# Autodesk Inventor assembly: mount3
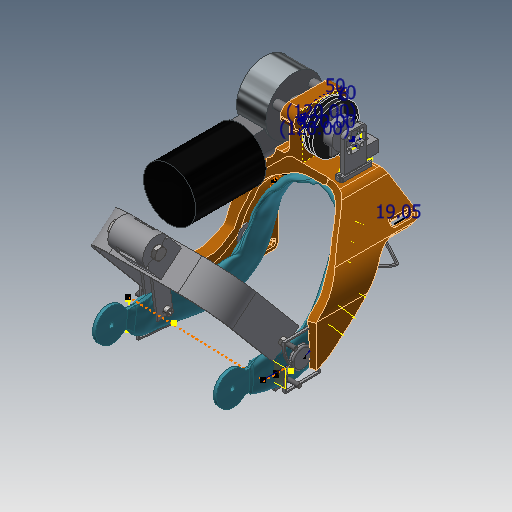
[picture p0: Inventor's stored thumbnail of the model, 512x512]
Saved by Autodesk Inventor 2025.2 (Build 292293000, 293)
## iProperties
Created: 2025-02-11
Part Number: mount3
Document SubType Name: Assembly
Designer: Alex
Author: Alex
## Documents named in this file (13)
- C:\Users\email\Desktop\Projects\Capstone\4TB6\CAD_Model\thigh_mount_2\mount3.iam
- C:\Users\email\Desktop\Projects\Capstone\4TB6\CAD_Model\thigh_mount_2\thigh.ipt
- C:\Users\email\Desktop\Projects\Capstone\4TB6\CAD_Model\thigh_mount_2\mount3.ipt
- C:\Users\email\Desktop\Projects\Capstone\4TB6\CAD_Model\thigh_mount_2\mount4.ipt
- C:\Users\email\Desktop\Projects\Capstone\4TB6\CAD_Model\thigh_mount_2\motor.ipt
- C:\Users\email\Desktop\Projects\Capstone\4TB6\CAD_Model\thigh_mount_2\spool_temp.ipt
- C:\Users\email\Desktop\Projects\Capstone\4TB6\CAD_Model\thigh_mount_2\magnetholder.ipt
- C:\Users\email\Desktop\Projects\Capstone\4TB6\CAD_Model\thigh_mount_2\imu_house_assembly.iam
- C:\Users\email\Desktop\Projects\Capstone\4TB6\CAD_Model\thigh_mount_2\ANSI B18.6.7M - M6x1 x 13(6).ipt
- C:\Users\email\Desktop\Projects\Capstone\4TB6\CAD_Model\thigh_mount_2\as5600mount_2.ipt
- C:\Users\email\Desktop\Projects\Capstone\4TB6\CAD_Model\thigh_mount_2\pulley_bracket_assem.iam
- C:\Users\email\Desktop\Projects\Capstone\4TB6\CAD_Model\thigh_mount_2\brace_tabs.ipt
- C:\Users\email\Desktop\Projects\Capstone\4TB6\CAD_Model\thigh_mount_2\brace_tabs_half.ipt
## Components (14 placed, 12 different names)
1. thigh:1 — Mate:1, Mate:2, Flush:1, Flush:2, Mate:28, Mate:29, Mate:30, Mate:31, Mate:32, Mate:33, Mate:34
2. mount3:1 — Flush:2
3. mount4:1 — Flush:4, Mate:3, Mate:4, Mate:5, Mate:12, Mate:13, Flush:5, Angle:7, Angle:2, Mate:21, Mate:22, Mate:27
4. motor:1 — Mate:3, Mate:4, Mate:5, Mate:7, Mate:23, Mate:24
5. spool_temp:1 — Mate:7, Mate:9, Mate:10, Mate:11, Mate:23, Mate:24
6. magnetholder:1 — Mate:9, Mate:10, Mate:11, Mate:18, Mate:25, Mate:26
7. imu_house_assembly:1 [sub-assembly] — Mate:12, Mate:13, Flush:5, Mate:14, Mate:15
8. Square Recessed Pan Head Machine Screw - Type III - Metric M6x1 x 13:1 — Mate:14, Mate:15
9. as5600mount_2:1 — Mate:18, Mate:25, Mate:26, Mate:27
10. pulley_bracket_assem:1 [sub-assembly] — Angle:7, Angle:2, Mate:21, Mate:22
11. brace_tabs:1 — Mate:28, Mate:29
12. brace_tabs:2 — Mate:30, Mate:31
13. brace_tabs_half:1 — Mate:32
14. brace_tabs_half:2 — Mate:33, Mate:34
## Relationships (35: Mate 28, Flush 5, Angle 2)
- Mate:1: thigh:1
- Mate:2: thigh:1
- Flush:1: thigh:1
- Flush:2: thigh:1 ↔ mount3:1
- Flush:3 (-15 mm)
- Flush:4: mount4:1
- Mate:3: mount4:1 ↔ motor:1
- Mate:4: mount4:1 ↔ motor:1
- Mate:5: mount4:1 ↔ motor:1
- Mate:7: motor:1 ↔ spool_temp:1
- Mate:9: spool_temp:1 ↔ magnetholder:1
- Mate:10: spool_temp:1 ↔ magnetholder:1
- Mate:11: spool_temp:1 ↔ magnetholder:1
- Mate:12: mount4:1 ↔ imu_house_assembly:1
- Mate:13: mount4:1 ↔ imu_house_assembly:1
- Flush:5: mount4:1 ↔ imu_house_assembly:1
- Mate:14: imu_house_assembly:1 ↔ Square Recessed Pan Head Machine Screw - Type III - Metric M6x1 x 13:1
- Mate:15: imu_house_assembly:1 ↔ Square Recessed Pan Head Machine Screw - Type III - Metric M6x1 x 13:1
- Mate:18: magnetholder:1 ↔ as5600mount_2:1
- Angle:7 (0 deg): mount4:1 ↔ pulley_bracket_assem:1
- Angle:2 (-40 deg): mount4:1 ↔ pulley_bracket_assem:1
- Mate:21 (-30 mm): mount4:1 ↔ pulley_bracket_assem:1
- Mate:22 (-40 mm): mount4:1 ↔ pulley_bracket_assem:1
- Mate:23: motor:1 ↔ spool_temp:1
- Mate:24: motor:1 ↔ spool_temp:1
- Mate:25: magnetholder:1 ↔ as5600mount_2:1
- Mate:26 (8 mm): magnetholder:1 ↔ as5600mount_2:1
- Mate:27: mount4:1 ↔ as5600mount_2:1
- Mate:28: thigh:1 ↔ brace_tabs:1
- Mate:29: thigh:1 ↔ brace_tabs:1
- Mate:30: thigh:1 ↔ brace_tabs:2
- Mate:31: thigh:1 ↔ brace_tabs:2
- Mate:32: thigh:1 ↔ brace_tabs_half:1
- Mate:33 (2 mm): thigh:1 ↔ brace_tabs_half:2
- Mate:34: thigh:1 ↔ brace_tabs_half:2
